# Autodesk Inventor assembly: femaleHeaders
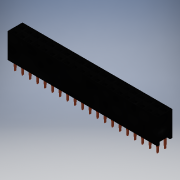
[picture p0: Inventor's stored thumbnail of the model, 180x180]
Saved by Autodesk Inventor 2016 (Build 200138000, 138)
## iProperties
Created: 2013-10-10
Part Number: femaleHeaders
Description: STEP AP203
Document SubType Name: Assembly
Designer: Jonathan
Sending System: SolidWorks 2012
Preprocessor: SwSTEP 2.0
Title: 960240-6202-AR.STEP
Revision Number: ANY
## Documents named in this file (3)
- C:\Users\Jonathan\Documents\Projects\anodePiShield\coincidenceCounter\cad\electronics\femaleHeaders\femaleHeaders.iam
- C:\Users\Jonathan\Documents\Projects\anodePiShield\coincidenceCounter\cad\electronics\femaleHeaders\960240-6202-AR Body.ipt
- C:\Users\Jonathan\Documents\Projects\anodePiShield\coincidenceCounter\cad\electronics\femaleHeaders\960240-6202-AR Pin.ipt
## Components (41 placed, 3 different names)
1. 960240-6202-AR Body_1 — Mate:1, Mate:2, Mate:3
2. 960240-6202-AR Pin_2 — Mate:1, Mate:2, Mate:3
3. 960240-6202-AR Pin:2
4. 960240-6202-AR Pin:3
5. 960240-6202-AR Pin:4
6. 960240-6202-AR Pin:5
7. 960240-6202-AR Pin:6
8. 960240-6202-AR Pin:7
9. 960240-6202-AR Pin:8
10. 960240-6202-AR Pin:9
11. 960240-6202-AR Pin:10
12. 960240-6202-AR Pin:11
13. 960240-6202-AR Pin:12
14. 960240-6202-AR Pin:13
15. 960240-6202-AR Pin:14
16. 960240-6202-AR Pin:15
17. 960240-6202-AR Pin:16
18. 960240-6202-AR Pin:17
19. 960240-6202-AR Pin:18
20. 960240-6202-AR Pin:19
21. 960240-6202-AR Pin:20
22. 960240-6202-AR Pin:21
23. 960240-6202-AR Pin:22
24. 960240-6202-AR Pin:23
25. 960240-6202-AR Pin:24
26. 960240-6202-AR Pin:25
27. 960240-6202-AR Pin:26
28. 960240-6202-AR Pin:27
29. 960240-6202-AR Pin:28
30. 960240-6202-AR Pin:29
31. 960240-6202-AR Pin:30
32. 960240-6202-AR Pin:31
33. 960240-6202-AR Pin:32
34. 960240-6202-AR Pin:33
35. 960240-6202-AR Pin:34
36. 960240-6202-AR Pin:35
37. 960240-6202-AR Pin:36
38. 960240-6202-AR Pin:37
39. 960240-6202-AR Pin:38
40. 960240-6202-AR Pin:39
41. 960240-6202-AR Pin:40
## Component patterns: (40 elements, first: 960240-6202-AR Pin_2)
## Relationships (3: Mate 3)
- Mate:1: 960240-6202-AR Body_1 ↔ 960240-6202-AR Pin_2
- Mate:2: 960240-6202-AR Body_1 ↔ 960240-6202-AR Pin_2
- Mate:3: 960240-6202-AR Body_1 ↔ 960240-6202-AR Pin_2
